# Autodesk Inventor assembly: mobile_robot_car
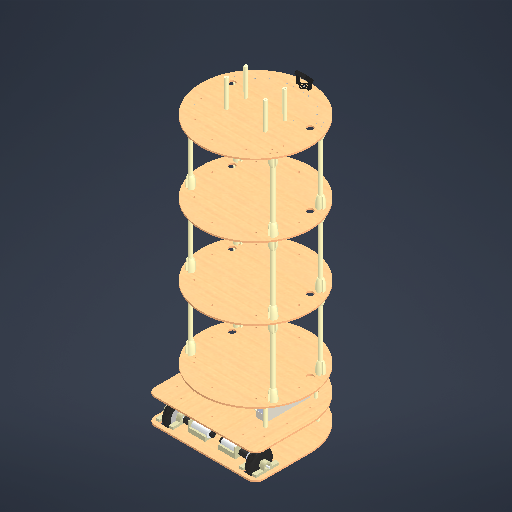
[picture p0: Inventor's stored thumbnail of the model, 512x512]
Saved by Autodesk Inventor 2026 (Build 300175050, 175E)
## iProperties
Created: 2025-06-05
Part Number: mobile_robot_car
Document SubType Name: Assembly
Designer: satom
Author: satom
## Documents named in this file (25)
- C:\Users\satom\Desktop\Robot\CAD\Inventor\mobile_robot_car.iam
- C:\Users\satom\Desktop\Robot\CAD\Inventor\C - Chassis\layer1_new.ipt
- C:\Users\satom\Desktop\Robot\CAD\Inventor\D - DriveTrain\motor_holder.ipt
- C:\Users\satom\Desktop\Robot\CAD\Inventor\D - DriveTrain\wheel_bearing.ipt
- C:\Users\satom\Desktop\Robot\CAD\Inventor\D - DriveTrain\wheel_mount.ipt
- C:\Users\satom\Desktop\Robot\CAD\Inventor\C - Chassis\3inch_standoff.ipt
- C:\Users\satom\Desktop\Robot\CAD\Inventor\solidworks\D - DriveTrain\ball_caster\ball_caster\ball_caster.ipt
- C:\Users\satom\Desktop\Robot\CAD\Inventor\solidworks\D - DriveTrain\motor\motor\motor.ipt
- C:\Users\satom\Desktop\Robot\CAD\Inventor\solidworks\D - DriveTrain\shaft_coupler\shaft_coupler\shaft_coupler.ipt
- C:\Users\satom\Desktop\Robot\CAD\Inventor\solidworks\D - DriveTrain\drive_shaft\drive_shaft\drive_shaft.ipt
- C:\Users\satom\Desktop\Robot\CAD\Inventor\solidworks\D - DriveTrain\ball_bearing\ball_bearing\ball_bearing.ipt
- C:\Users\satom\Desktop\Robot\CAD\Inventor\solidworks\D - DriveTrain\wheel\wheel\wheel.ipt
- C:\Users\satom\Desktop\Robot\CAD\Inventor\solidworks\E - Electronics\Main Board\Main Board\Main Board.ipt
- C:\Users\satom\Desktop\Robot\CAD\Inventor\solidworks\E - Electronics\NiMH_battery\NiMH_battery\NiMH_battery.ipt
- C:\Users\satom\Desktop\Robot\CAD\Inventor\solidworks\C - Chassis\NiMH_holder\NiMH_holder\NiMH_holder.ipt
- C:\Users\satom\Desktop\Robot\CAD\Inventor\C - Chassis\layer2_new.ipt
- C:\Users\satom\Desktop\Robot\CAD\Inventor\solidworks\E - Electronics\IMU breakout\IMU breakout\IMU breakout.ipt
- C:\Users\satom\Desktop\Robot\CAD\Inventor\solidworks\E - Electronics\jetson_orin_nano_platform\jetson_orin_nano_platform\jetson_orin_nano_platform.ipt
- C:\Users\satom\Desktop\Robot\CAD\Inventor\C - Chassis\layer3_new.ipt
- C:\Users\satom\Desktop\Robot\CAD\Inventor\C - Chassis\9inch_spacer.ipt
- C:\Users\satom\Desktop\Robot\CAD\Inventor\C - Chassis\layer4_new.ipt
- C:\Users\satom\Desktop\Robot\CAD\Inventor\C - Chassis\layer5_new.ipt
- C:\Users\satom\Desktop\Robot\CAD\Inventor\C - Chassis\layer6_new.ipt
- C:\Users\satom\Desktop\Robot\CAD\Inventor\C - Chassis\3.5inch_standoff.ipt
- C:\Users\satom\Desktop\Robot\CAD\Inventor\solidworks\Display\Arducam_assembly\Arducam_assembly\Arducam_assembly.ipt
## Components (61 placed, 24 different names)
1. layer1_new:1 — Mate:1, Mate:2, Mate:3, Mate:4, Mate:5, Mate:6, Mate:8, Mate:9, Mate:10, Mate:11, Mate:12, Mate:13, Mate:14, Mate:15, Mate:18, Mate:19, Mate:20, Mate:21, Mate:22, Mate:23, Mate:24, Mate:25, Mate:26, Mate:27, Mate:28, Mate:33, Mate:34, Mate:65, Mate:66, Mate:67
2. motor_holder:1 — Mate:1, Mate:29, Mate:30, Mate:34
3. motor_holder:2 — Mate:2, Mate:31, Mate:32, Mate:33
4. wheel_bearing:1 — Mate:5, Mate:12, Mate:13, Mate:43, Mate:44
5. wheel_bearing:2 — Mate:6, Mate:10, Mate:11, Mate:50, Mate:51
6. wheel_bearing:3 — Mate:4, Mate:14, Mate:15, Mate:45, Mate:46
7. wheel_bearing:4 — Mate:3, Mate:8, Mate:9, Mate:48, Mate:49
8. wheel_mount:1 — Mate:55, Mate:56, Mate:62
9. wheel_mount:2 — Mate:57, Mate:58, Mate:64
10. wheel_mount:3 — Mate:53, Mate:54
11. wheel_mount:4 — Mate:59, Mate:60, Mate:61, Mate:63
12. 3inch_standoff:1 — Mate:18, Mate:24, Mate:82
13. 3inch_standoff:2 — Mate:19, Mate:25, Mate:79, Mate:81
14. 3inch_standoff:3 — Mate:21, Mate:23, Mate:83
15. 3inch_standoff:4 — Mate:20, Mate:22, Mate:80
16. ball_caster:1 — Mate:26, Mate:27, Mate:28
17. motor:1 — Mate:29, Mate:30, Mate:35, Mate:37
18. motor:2 — Mate:31, Mate:32, Mate:36, Mate:38
19. shaft_coupler:1 — Mate:36, Mate:38, Mate:39, Mate:41
20. shaft_coupler:2 — Mate:35, Mate:37, Mate:40, Mate:42
21. drive_shaft:1 — Mate:39, Mate:41, Mate:62
22. drive_shaft:2 — Mate:40, Mate:42, Mate:61
23. ball_bearing:1 — Mate:50, Mate:51
24. ball_bearing:2 — Mate:45, Mate:46
25. ball_bearing:3 — Mate:43, Mate:44, Mate:63
26. ball_bearing:4 — Mate:48, Mate:49, Mate:64
27. wheel:1 — Mate:55, Mate:56, Mate:57, Mate:58
28. wheel:2 — Mate:53, Mate:54, Mate:59, Mate:60
29. Main Board:1 — Mate:65, Mate:66, Mate:67
30. NiMH_battery:1 — Mate:76, Mate:77
31. NiMH_battery:2 — Mate:74, Mate:78
32. NiMH_holder:1 — Mate:74, Mate:78, Mate:84, Mate:86, Mate:87
33. NiMH_holder:2 — Mate:76, Mate:77, Mate:85, Mate:88, Mate:89
34. layer2_new:1 — Mate:79, Mate:80, Mate:81, Mate:82, Mate:83, Mate:84, Mate:85, Mate:86, Mate:87, Mate:88, Mate:89, Mate:90, Mate:91, Mate:92, Mate:93, Mate:94, Mate:95, Mate:96, Mate:97, Mate:98, Mate:99, Mate:100, Mate:101, Mate:102
35. IMU breakout:1 — Mate:90, Mate:91, Mate:92
36. jetson_orin_nano_platform:1 — Mate:93, Mate:94
37. 3inch_standoff:5 — Mate:97, Mate:101, Mate:103, Mate:104
38. 3inch_standoff:6 — Mate:96, Mate:102
39. 3inch_standoff:7 — Mate:98, Mate:99
40. 3inch_standoff:8 — Mate:95, Mate:100, Mate:105
41. layer3_new:1 — Mate:103, Mate:104, Mate:105, Mate:106, Mate:107, Mate:108, Mate:109, Mate:110, Mate:111, Mate:112, Mate:113, Mate:114, Mate:115, Mate:116, Mate:117, Mate:118, Mate:119, Mate:120, Mate:121
42. 9inch_spacer:1 — Mate:106, Mate:116, Mate:117, Mate:118, Mate:126, Mate:127
43. 9inch_spacer:2 — Mate:107, Mate:119, Mate:120, Mate:121, Mate:122, Mate:123, Mate:124, Mate:125
44. 9inch_spacer:3 — Mate:108, Mate:110, Mate:111, Mate:112, Mate:130, Mate:131
45. 9inch_spacer:4 — Mate:109, Mate:113, Mate:114, Mate:115, Mate:128, Mate:129
46. layer4_new:1 — Mate:122, Mate:123, Mate:124, Mate:125, Mate:126, Mate:127, Mate:128, Mate:129, Mate:130, Mate:131, Mate:132, Mate:133, Mate:134, Mate:135, Mate:136, Mate:137, Mate:138, Mate:139, Mate:140, Mate:141, Mate:142, Mate:143, Mate:144, Mate:145, Mate:146, Mate:147
47. 9inch_spacer:5 — Mate:135, Mate:145, Mate:146, Mate:147, Mate:148, Mate:152, Mate:153, Mate:154
48. 9inch_spacer:6 — Mate:134, Mate:142, Mate:143, Mate:144, Mate:155, Mate:156, Mate:157
49. 9inch_spacer:7 — Mate:133, Mate:136, Mate:137, Mate:138, Mate:158, Mate:159, Mate:160
50. 9inch_spacer:8 — Mate:132, Mate:139, Mate:140, Mate:141, Mate:149, Mate:150, Mate:151
51. layer5_new:1 — Mate:148, Mate:149, Mate:150, Mate:151, Mate:152, Mate:153, Mate:154, Mate:155, Mate:156, Mate:157, Mate:158, Mate:159, Mate:160, Mate:161, Mate:162, Mate:163, Mate:164, Mate:165, Mate:166, Mate:167, Mate:168, Mate:169, Mate:170, Mate:171, Mate:172, Mate:173, Mate:174, Mate:175, Mate:176
52. 9inch_spacer:9 — Mate:161, Mate:171, Mate:172, Mate:173, Mate:177, Mate:178, Mate:179, Mate:180
53. 9inch_spacer:10 — Mate:162, Mate:174, Mate:175, Mate:176, Mate:181, Mate:182, Mate:183
54. 9inch_spacer:11 — Mate:163, Mate:168, Mate:169, Mate:170, Mate:187, Mate:188, Mate:189
55. 9inch_spacer:12 — Mate:164, Mate:165, Mate:166, Mate:167, Mate:184, Mate:185, Mate:186
56. layer6_new:1 — Mate:177, Mate:178, Mate:179, Mate:180, Mate:181, Mate:182, Mate:183, Mate:184, Mate:185, Mate:186, Mate:187, Mate:188, Mate:189, Mate:190, Mate:191, Mate:192, Mate:193, Mate:194, Mate:195, Mate:196, Mate:197, Mate:198, Mate:199
57. 3.5inch_standoff:1 — Mate:191, Mate:194
58. 3.5inch_standoff:2 — Mate:190, Mate:197
59. 3.5inch_standoff:3 — Mate:192, Mate:196
60. 3.5inch_standoff:4 — Mate:193, Mate:195
61. Arducam_assembly:1 — Mate:198, Mate:199
## Relationships (187: Mate 187)
- Mate:1: layer1_new:1 ↔ motor_holder:1
- Mate:2: layer1_new:1 ↔ motor_holder:2
- Mate:3: layer1_new:1 ↔ wheel_bearing:4
- Mate:4: layer1_new:1 ↔ wheel_bearing:3
- Mate:5: layer1_new:1 ↔ wheel_bearing:1
- Mate:6: layer1_new:1 ↔ wheel_bearing:2
- Mate:8: layer1_new:1 ↔ wheel_bearing:4
- Mate:9: layer1_new:1 ↔ wheel_bearing:4
- Mate:10: layer1_new:1 ↔ wheel_bearing:2
- Mate:11: layer1_new:1 ↔ wheel_bearing:2
- Mate:12: layer1_new:1 ↔ wheel_bearing:1
- Mate:13: layer1_new:1 ↔ wheel_bearing:1
- Mate:14: layer1_new:1 ↔ wheel_bearing:3
- Mate:15: layer1_new:1 ↔ wheel_bearing:3
- Mate:18: layer1_new:1 ↔ 3inch_standoff:1
- Mate:19: layer1_new:1 ↔ 3inch_standoff:2
- Mate:20: layer1_new:1 ↔ 3inch_standoff:4
- Mate:21: layer1_new:1 ↔ 3inch_standoff:3
- Mate:22: layer1_new:1 ↔ 3inch_standoff:4
- Mate:23: layer1_new:1 ↔ 3inch_standoff:3
- Mate:24: layer1_new:1 ↔ 3inch_standoff:1
- Mate:25: layer1_new:1 ↔ 3inch_standoff:2
- Mate:26: layer1_new:1 ↔ ball_caster:1
- Mate:27: layer1_new:1 ↔ ball_caster:1
- Mate:28: layer1_new:1 ↔ ball_caster:1
- Mate:29: motor_holder:1 ↔ motor:1
- Mate:30: motor_holder:1 ↔ motor:1
- Mate:31: motor_holder:2 ↔ motor:2
- Mate:32: motor_holder:2 ↔ motor:2
- Mate:33: layer1_new:1 ↔ motor_holder:2
- Mate:34: layer1_new:1 ↔ motor_holder:1
- Mate:35: motor:1 ↔ shaft_coupler:2
- Mate:36: motor:2 ↔ shaft_coupler:1
- Mate:37 (0.508 mm): motor:1 ↔ shaft_coupler:2
- Mate:38 (0.508 mm): motor:2 ↔ shaft_coupler:1
- Mate:39: shaft_coupler:1 ↔ drive_shaft:1
- Mate:40: shaft_coupler:2 ↔ drive_shaft:2
- Mate:41: shaft_coupler:1 ↔ drive_shaft:1
- Mate:42: shaft_coupler:2 ↔ drive_shaft:2
- Mate:43: wheel_bearing:1 ↔ ball_bearing:3
- Mate:44: wheel_bearing:1 ↔ ball_bearing:3
- Mate:45: wheel_bearing:3 ↔ ball_bearing:2
- Mate:46: wheel_bearing:3 ↔ ball_bearing:2
- Mate:48: wheel_bearing:4 ↔ ball_bearing:4
- Mate:49: wheel_bearing:4 ↔ ball_bearing:4
- Mate:50: wheel_bearing:2 ↔ ball_bearing:1
- Mate:51: wheel_bearing:2 ↔ ball_bearing:1
- Mate:53: wheel_mount:3 ↔ wheel:2
- Mate:54: wheel_mount:3 ↔ wheel:2
- Mate:55: wheel_mount:1 ↔ wheel:1
- Mate:56: wheel_mount:1 ↔ wheel:1
- Mate:57: wheel_mount:2 ↔ wheel:1
- Mate:58: wheel_mount:2 ↔ wheel:1
- Mate:59: wheel_mount:4 ↔ wheel:2
- Mate:60: wheel_mount:4 ↔ wheel:2
- Mate:61: wheel_mount:4 ↔ drive_shaft:2
- Mate:62: wheel_mount:1 ↔ drive_shaft:1
- Mate:63 (2.54 mm): wheel_mount:4 ↔ ball_bearing:3
- Mate:64 (2.54 mm): wheel_mount:2 ↔ ball_bearing:4
- Mate:65: layer1_new:1 ↔ Main Board:1
- Mate:66: layer1_new:1 ↔ Main Board:1
- Mate:67: layer1_new:1 ↔ Main Board:1
- Mate:74: NiMH_battery:2 ↔ NiMH_holder:1
- Mate:76: NiMH_battery:1 ↔ NiMH_holder:2
- Mate:77: NiMH_battery:1 ↔ NiMH_holder:2
- Mate:78: NiMH_battery:2 ↔ NiMH_holder:1
- Mate:79: 3inch_standoff:2 ↔ layer2_new:1
- Mate:80: 3inch_standoff:4 ↔ layer2_new:1
- Mate:81: 3inch_standoff:2 ↔ layer2_new:1
- Mate:82: 3inch_standoff:1 ↔ layer2_new:1
- Mate:83: 3inch_standoff:3 ↔ layer2_new:1
- Mate:84: NiMH_holder:1 ↔ layer2_new:1
- Mate:85: NiMH_holder:2 ↔ layer2_new:1
- Mate:86: NiMH_holder:1 ↔ layer2_new:1
- Mate:87: NiMH_holder:1 ↔ layer2_new:1
- Mate:88: NiMH_holder:2 ↔ layer2_new:1
- Mate:89: NiMH_holder:2 ↔ layer2_new:1
- Mate:90: layer2_new:1 ↔ IMU breakout:1
- Mate:91: layer2_new:1 ↔ IMU breakout:1
- Mate:92: layer2_new:1 ↔ IMU breakout:1
- Mate:93: layer2_new:1 ↔ jetson_orin_nano_platform:1
- Mate:94: layer2_new:1 ↔ jetson_orin_nano_platform:1
- Mate:95: layer2_new:1 ↔ 3inch_standoff:8
- Mate:96: layer2_new:1 ↔ 3inch_standoff:6
- Mate:97: layer2_new:1 ↔ 3inch_standoff:5
- Mate:98: layer2_new:1 ↔ 3inch_standoff:7
- Mate:99: layer2_new:1 ↔ 3inch_standoff:7
- Mate:100: layer2_new:1 ↔ 3inch_standoff:8
- Mate:101: layer2_new:1 ↔ 3inch_standoff:5
- Mate:102: layer2_new:1 ↔ 3inch_standoff:6
- Mate:103: 3inch_standoff:5 ↔ layer3_new:1
- Mate:104: 3inch_standoff:5 ↔ layer3_new:1
- Mate:105: 3inch_standoff:8 ↔ layer3_new:1
- Mate:106: layer3_new:1 ↔ 9inch_spacer:1
- Mate:107: layer3_new:1 ↔ 9inch_spacer:2
- Mate:108: layer3_new:1 ↔ 9inch_spacer:3
- Mate:109: layer3_new:1 ↔ 9inch_spacer:4
- Mate:110: layer3_new:1 ↔ 9inch_spacer:3
- Mate:111: layer3_new:1 ↔ 9inch_spacer:3
- Mate:112: layer3_new:1 ↔ 9inch_spacer:3
- Mate:113: layer3_new:1 ↔ 9inch_spacer:4
- Mate:114: layer3_new:1 ↔ 9inch_spacer:4
- Mate:115: layer3_new:1 ↔ 9inch_spacer:4
- Mate:116: layer3_new:1 ↔ 9inch_spacer:1
- Mate:117: layer3_new:1 ↔ 9inch_spacer:1
- Mate:118: layer3_new:1 ↔ 9inch_spacer:1
- Mate:119: layer3_new:1 ↔ 9inch_spacer:2
- Mate:120: layer3_new:1 ↔ 9inch_spacer:2
- Mate:121: layer3_new:1 ↔ 9inch_spacer:2
- Mate:122: 9inch_spacer:2 ↔ layer4_new:1
- Mate:123: 9inch_spacer:2 ↔ layer4_new:1
- Mate:124: 9inch_spacer:2 ↔ layer4_new:1
- Mate:125: 9inch_spacer:2 ↔ layer4_new:1
- Mate:126: 9inch_spacer:1 ↔ layer4_new:1
- Mate:127: 9inch_spacer:1 ↔ layer4_new:1
- Mate:128: 9inch_spacer:4 ↔ layer4_new:1
- Mate:129: 9inch_spacer:4 ↔ layer4_new:1
- Mate:130: 9inch_spacer:3 ↔ layer4_new:1
- Mate:131: 9inch_spacer:3 ↔ layer4_new:1
- Mate:132: layer4_new:1 ↔ 9inch_spacer:8
- Mate:133: layer4_new:1 ↔ 9inch_spacer:7
- Mate:134: layer4_new:1 ↔ 9inch_spacer:6
- Mate:135: layer4_new:1 ↔ 9inch_spacer:5
- Mate:136: layer4_new:1 ↔ 9inch_spacer:7
- Mate:137: layer4_new:1 ↔ 9inch_spacer:7
- Mate:138: layer4_new:1 ↔ 9inch_spacer:7
- Mate:139: layer4_new:1 ↔ 9inch_spacer:8
- Mate:140: layer4_new:1 ↔ 9inch_spacer:8
- Mate:141: layer4_new:1 ↔ 9inch_spacer:8
- Mate:142: layer4_new:1 ↔ 9inch_spacer:6
- Mate:143: layer4_new:1 ↔ 9inch_spacer:6
- Mate:144: layer4_new:1 ↔ 9inch_spacer:6
- Mate:145: layer4_new:1 ↔ 9inch_spacer:5
- Mate:146: layer4_new:1 ↔ 9inch_spacer:5
- Mate:147: layer4_new:1 ↔ 9inch_spacer:5
- Mate:148: 9inch_spacer:5 ↔ layer5_new:1
- Mate:149: 9inch_spacer:8 ↔ layer5_new:1
- Mate:150: 9inch_spacer:8 ↔ layer5_new:1
- Mate:151: 9inch_spacer:8 ↔ layer5_new:1
- Mate:152: 9inch_spacer:5 ↔ layer5_new:1
- Mate:153: 9inch_spacer:5 ↔ layer5_new:1
- Mate:154: 9inch_spacer:5 ↔ layer5_new:1
- Mate:155: 9inch_spacer:6 ↔ layer5_new:1
- Mate:156: 9inch_spacer:6 ↔ layer5_new:1
- Mate:157: 9inch_spacer:6 ↔ layer5_new:1
- Mate:158: 9inch_spacer:7 ↔ layer5_new:1
- Mate:159: 9inch_spacer:7 ↔ layer5_new:1
- Mate:160: 9inch_spacer:7 ↔ layer5_new:1
- Mate:161: layer5_new:1 ↔ 9inch_spacer:9
- Mate:162: layer5_new:1 ↔ 9inch_spacer:10
- Mate:163: layer5_new:1 ↔ 9inch_spacer:11
- Mate:164: layer5_new:1 ↔ 9inch_spacer:12
- Mate:165: layer5_new:1 ↔ 9inch_spacer:12
- Mate:166: layer5_new:1 ↔ 9inch_spacer:12
- Mate:167: layer5_new:1 ↔ 9inch_spacer:12
- Mate:168: layer5_new:1 ↔ 9inch_spacer:11
- Mate:169: layer5_new:1 ↔ 9inch_spacer:11
- Mate:170: layer5_new:1 ↔ 9inch_spacer:11
- Mate:171: layer5_new:1 ↔ 9inch_spacer:9
- Mate:172: layer5_new:1 ↔ 9inch_spacer:9
- Mate:173: layer5_new:1 ↔ 9inch_spacer:9
- Mate:174: layer5_new:1 ↔ 9inch_spacer:10
- Mate:175: layer5_new:1 ↔ 9inch_spacer:10
- Mate:176: layer5_new:1 ↔ 9inch_spacer:10
- Mate:177: 9inch_spacer:9 ↔ layer6_new:1
- Mate:178: 9inch_spacer:9 ↔ layer6_new:1
- Mate:179: 9inch_spacer:9 ↔ layer6_new:1
- Mate:180: 9inch_spacer:9 ↔ layer6_new:1
- Mate:181: 9inch_spacer:10 ↔ layer6_new:1
- Mate:182: 9inch_spacer:10 ↔ layer6_new:1
- Mate:183: 9inch_spacer:10 ↔ layer6_new:1
- Mate:184: 9inch_spacer:12 ↔ layer6_new:1
- Mate:185: 9inch_spacer:12 ↔ layer6_new:1
- Mate:186: 9inch_spacer:12 ↔ layer6_new:1
- Mate:187: 9inch_spacer:11 ↔ layer6_new:1
- Mate:188: 9inch_spacer:11 ↔ layer6_new:1
- Mate:189: 9inch_spacer:11 ↔ layer6_new:1
- Mate:190: layer6_new:1 ↔ 3.5inch_standoff:2
- Mate:191: layer6_new:1 ↔ 3.5inch_standoff:1
- Mate:192: layer6_new:1 ↔ 3.5inch_standoff:3
- Mate:193: layer6_new:1 ↔ 3.5inch_standoff:4
- Mate:194: layer6_new:1 ↔ 3.5inch_standoff:1
- Mate:195: layer6_new:1 ↔ 3.5inch_standoff:4
- Mate:196: layer6_new:1 ↔ 3.5inch_standoff:3
- Mate:197: layer6_new:1 ↔ 3.5inch_standoff:2
- Mate:198: layer6_new:1 ↔ Arducam_assembly:1
- Mate:199: layer6_new:1 ↔ Arducam_assembly:1
## Named parameters: m3_heat_set_insert = 4 mm
